# Autodesk Inventor assembly: extruder assembly_MIR
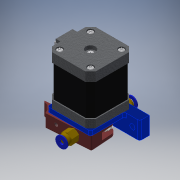
[picture p0: Inventor's stored thumbnail of the model, 180x180]
Saved by Autodesk Inventor 2016 SP1 (Build 200210100, 210)
## iProperties
Created: 2015-12-27
Part Number: extruder assembly_MIR
Document SubType Name: Assembly
Designer: ubik
Author: Dirk Alferink
## Documents named in this file (7)
- E:\GitHub\kossel-XXL\extruder assembly_MIR.iam
- E:\GitHub\kossel-XXL\Part1_MIR1.ipt
- E:\GitHub\kossel-XXL\Part2_MIR1.ipt
- C:\Users\ubik\Dropbox\proiecte\inventor\kossel\NEMA17 Stepper_MIR.ipt
- C:\Users\ubik\Dropbox\proiecte\inventor\kossel\Bowden_MIR.ipt
- E:\GitHub\kossel-XXL\Drive Gear_MIR.ipt
- E:\GitHub\kossel-XXL\idler bearing_MIR.ipt
## Components (7 placed, 6 different names)
1. Part1_MIR1:1 — Insert:3, Insert:2, Insert:1, Insert:5
2. Part2_MIR1:1 — Insert:3, Insert:4, Insert:13
3. NEMA17 Stepper_MIR:1 — Insert:2, Insert:1, Insert:6
4. Bowden_MIR:1 — Insert:4
5. Bowden_MIR:2 — Insert:5
6. Drive Gear_MIR:1 — Insert:6
7. idler bearing_MIR:1 — Insert:13
## Relationships (7: Insert 7)
- Insert:3: Part1_MIR1:1 ↔ Part2_MIR1:1
- Insert:2: Part1_MIR1:1 ↔ NEMA17 Stepper_MIR:1
- Insert:1: Part1_MIR1:1 ↔ NEMA17 Stepper_MIR:1
- Insert:4: Part2_MIR1:1 ↔ Bowden_MIR:1
- Insert:5: Part1_MIR1:1 ↔ Bowden_MIR:2
- Insert:6 (1 mm): NEMA17 Stepper_MIR:1 ↔ Drive Gear_MIR:1
- Insert:13: Part2_MIR1:1 ↔ idler bearing_MIR:1
